# Autodesk Inventor assembly: LR_01
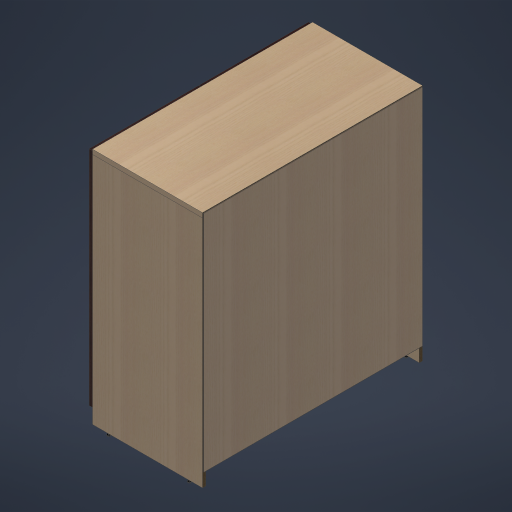
[picture p0: Inventor's stored thumbnail of the model, 512x512]
Saved by Autodesk Inventor 2024.3 (Build 283343000, 343)
## iProperties
Created: 2013-04-03
Part Number: LR_01
Document SubType Name: Assembly
Designer: User
Description: Coat Check
Material Code: Item.FillWorkpiece.Material.Code
Author: User
## Documents named in this file (17)
- C:\W4INV 2024 Design\PROJECTS\Living Room\Coat Check\LR_01.iam
- C:\W4INV 2024 Design\PROJECTS\Samples\Living Room\Coat Check\LR_0108.ipt
- C:\W4INV 2024 Design\PROJECTS\Samples\Living Room\Coat Check\LR_0103.ipt
- C:\W4INV 2024 Design\PROJECTS\Samples\Living Room\Coat Check\LR_0100.ipt
- C:\W4INV 2024 Design\PROJECTS\Samples\Living Room\Coat Check\LR_0102.ipt
- C:\W4INV 2024 Design\PROJECTS\Samples\Living Room\Coat Check\LR_0104.ipt
- C:\W4INV 2024 Design\PROJECTS\Samples\Living Room\Coat Check\LR_0101.ipt
- C:\W4INV 2024 Design\PROJECTS\Samples\Living Room\Coat Check\LR_0105.ipt
- C:\W4INV 2024 Design\PROJECTS\Samples\Living Room\Coat Check\LR_0106.ipt
- C:\W4INV 2024 Design\PROJECTS\Samples\Living Room\Coat Check\LR_0107.ipt
- C:\W4INV 2024 Design\_LIBRARY\Hinges\CONCEALED HINGE\Full Overlay Hinge Wood Screw Cup Wood Screw T18.iam
- C:\W4INV 2024 Design\_LIBRARY\Fixed joints\Minifix joint\MINIFIX D15 v2\Minifix D15 & Dowel L34 & Cap D15 PB T18 LH.ipt
- C:\W4INV 2024 Design\_LIBRARY\Fixed joints\Minifix joint\MINIFIX D15 v2\Minifix D15 & Dowel L34 & Cap D15 PB T18 RH.ipt
- C:\W4INV 2024 Design\_LIBRARY\Supports and legs\Supports\ADJUSTABLE SUPPORT\Support M6 H27 D18 with Bushing SB T18.ipt
- C:\W4INV 2023 Design\LIBRARY\Hinges\CONCEALED HINGE.iam
- C:\W4INV 2023 Design\LIBRARY\Supports and legs\Supports\ADJUSTABLE SUPPORT.ipt
- C:\W4INV 2023 Design\LIBRARY\Fixed joints\Minifix joint\MINIFIX D15 v2.ipt
## Components (29 placed, 13 different names)
1. LR_0108-Top:1 — Mate:46, Mate:48, Mate:50, Mate:52, Mate:54, Mate:56
2. LR_0103-Left Side:1 — Mate:14, Flush:30, Mate:16, Mate:18, Flush:32, Mate:20, Flush:33, Mate:22, Mate:24, Flush:35, Mate:26, Mate:28, Mate:30, Mate:38, Flush:45, Flush:48
3. LR_0100-Right Side:1 — Flush:1, Flush:2, Flush:29, Flush:31, Flush:34, Flush:36, Mate:36, Mate:44, Flush:47, Flush:50
4. LR_0102-Bottom:1 — Flush:37, Flush:40, Flush:41, Flush:44, Mate:58, Mate:60
5. LR_0104-Left Door:1
6. LR_0101-Right Door:1 — Flush:3, Flush:4
7. LR_0105-Back:1
8. LR_0106-Plynth:1
9. LR_0107-Vertical Partition:1 — Flush:46, Flush:49, Flush:51, Flush:52
10. Full Overlay Hinge Wood Screw Cup Wood Screw T18:1 [sub-assembly] — Mate:13, Flush:29, Mate:14
11. Full Overlay Hinge Wood Screw Cup Wood Screw T18:2 [sub-assembly] — Mate:15, Flush:30, Mate:16
12. Full Overlay Hinge Wood Screw Cup Wood Screw T18:3 [sub-assembly] — Mate:17, Flush:31, Mate:18
13. Full Overlay Hinge Wood Screw Cup Wood Screw T18:4 [sub-assembly] — Mate:19, Flush:32, Mate:20
14. Support M6 H27 D18 with Bushing SB T18:6 — Mate:21, Flush:33, Mate:22
15. Support M6 H27 D18 with Bushing SB T18:7 — Mate:23, Flush:34, Mate:24
16. Support M6 H27 D18 with Bushing SB T18:8 — Mate:25, Flush:35, Mate:26
17. Support M6 H27 D18 with Bushing SB T18:9 — Mate:27, Flush:36, Mate:28
18. Minifix D15 & Dowel L34 & Cap D15 PB T18 LH:1 — Mate:29, Mate:30, Flush:37
19. Minifix D15 & Dowel L34 & Cap D15 PB T18 RH:4 — Mate:35, Mate:36, Flush:40
20. Minifix D15 & Dowel L34 & Cap D15 PB T18 RH:5 — Mate:37, Mate:38, Flush:41
21. Minifix D15 & Dowel L34 & Cap D15 PB T18 LH:8 — Mate:43, Mate:44, Flush:44
22. Minifix D15 & Dowel L34 & Cap D15 PB T18 LH:9 — Mate:45, Flush:45, Mate:46
23. Minifix D15 & Dowel L34 & Cap D15 PB T18 RH:10 — Mate:47, Flush:46, Mate:48
24. Minifix D15 & Dowel L34 & Cap D15 PB T18 RH:11 — Mate:49, Flush:47, Mate:50
25. Minifix D15 & Dowel L34 & Cap D15 PB T18 RH:12 — Mate:51, Flush:48, Mate:52
26. Minifix D15 & Dowel L34 & Cap D15 PB T18 LH:13 — Mate:53, Flush:49, Mate:54
27. Minifix D15 & Dowel L34 & Cap D15 PB T18 LH:14 — Mate:55, Flush:50, Mate:56
28. Minifix D15 & Dowel L34 & Cap D15 PB T18 LH:15 — Mate:57, Mate:58, Flush:51
29. Minifix D15 & Dowel L34 & Cap D15 PB T18 RH:16 — Mate:59, Mate:60, Flush:52
## Relationships (64: Mate 40, Flush 24)
- Flush:1 (-80 mm): LR_0100-Right Side:1
- Flush:2 (-80 mm): LR_0100-Right Side:1
- Flush:3 (-100 mm): LR_0101-Right Door:1
- Flush:4 (-100 mm): LR_0101-Right Door:1
- Mate:13: Full Overlay Hinge Wood Screw Cup Wood Screw T18:1
- Flush:29: LR_0100-Right Side:1 ↔ Full Overlay Hinge Wood Screw Cup Wood Screw T18:1
- Mate:14: LR_0103-Left Side:1 ↔ Full Overlay Hinge Wood Screw Cup Wood Screw T18:1
- Mate:15: Full Overlay Hinge Wood Screw Cup Wood Screw T18:2
- Flush:30: LR_0103-Left Side:1 ↔ Full Overlay Hinge Wood Screw Cup Wood Screw T18:2
- Mate:16: LR_0103-Left Side:1 ↔ Full Overlay Hinge Wood Screw Cup Wood Screw T18:2
- Mate:17: Full Overlay Hinge Wood Screw Cup Wood Screw T18:3
- Flush:31: LR_0100-Right Side:1 ↔ Full Overlay Hinge Wood Screw Cup Wood Screw T18:3
- Mate:18: LR_0103-Left Side:1 ↔ Full Overlay Hinge Wood Screw Cup Wood Screw T18:3
- Mate:19: Full Overlay Hinge Wood Screw Cup Wood Screw T18:4
- Flush:32: LR_0103-Left Side:1 ↔ Full Overlay Hinge Wood Screw Cup Wood Screw T18:4
- Mate:20: LR_0103-Left Side:1 ↔ Full Overlay Hinge Wood Screw Cup Wood Screw T18:4
- Mate:21: Support M6 H27 D18 with Bushing SB T18:6
- Flush:33 (9 mm): LR_0103-Left Side:1 ↔ Support M6 H27 D18 with Bushing SB T18:6
- Mate:22 (17.5 mm): LR_0103-Left Side:1 ↔ Support M6 H27 D18 with Bushing SB T18:6
- Mate:23: Support M6 H27 D18 with Bushing SB T18:7
- Flush:34 (9 mm): LR_0100-Right Side:1 ↔ Support M6 H27 D18 with Bushing SB T18:7
- Mate:24 (17.5 mm): LR_0103-Left Side:1 ↔ Support M6 H27 D18 with Bushing SB T18:7
- Mate:25: Support M6 H27 D18 with Bushing SB T18:8
- Flush:35 (9 mm): LR_0103-Left Side:1 ↔ Support M6 H27 D18 with Bushing SB T18:8
- Mate:26 (17.5 mm): LR_0103-Left Side:1 ↔ Support M6 H27 D18 with Bushing SB T18:8
- Mate:27: Support M6 H27 D18 with Bushing SB T18:9
- Flush:36 (9 mm): LR_0100-Right Side:1 ↔ Support M6 H27 D18 with Bushing SB T18:9
- Mate:28 (17.5 mm): LR_0103-Left Side:1 ↔ Support M6 H27 D18 with Bushing SB T18:9
- Mate:29: Minifix D15 & Dowel L34 & Cap D15 PB T18 LH:1
- Mate:30: LR_0103-Left Side:1 ↔ Minifix D15 & Dowel L34 & Cap D15 PB T18 LH:1
- Flush:37 (18 mm): LR_0102-Bottom:1 ↔ Minifix D15 & Dowel L34 & Cap D15 PB T18 LH:1
- Mate:35: Minifix D15 & Dowel L34 & Cap D15 PB T18 RH:4
- Mate:36: LR_0100-Right Side:1 ↔ Minifix D15 & Dowel L34 & Cap D15 PB T18 RH:4
- Flush:40 (18 mm): LR_0102-Bottom:1 ↔ Minifix D15 & Dowel L34 & Cap D15 PB T18 RH:4
- Mate:37: Minifix D15 & Dowel L34 & Cap D15 PB T18 RH:5
- Mate:38: LR_0103-Left Side:1 ↔ Minifix D15 & Dowel L34 & Cap D15 PB T18 RH:5
- Flush:41 (18 mm): LR_0102-Bottom:1 ↔ Minifix D15 & Dowel L34 & Cap D15 PB T18 RH:5
- Mate:43: Minifix D15 & Dowel L34 & Cap D15 PB T18 LH:8
- Mate:44: LR_0100-Right Side:1 ↔ Minifix D15 & Dowel L34 & Cap D15 PB T18 LH:8
- Flush:44 (18 mm): LR_0102-Bottom:1 ↔ Minifix D15 & Dowel L34 & Cap D15 PB T18 LH:8
- Mate:45: Minifix D15 & Dowel L34 & Cap D15 PB T18 LH:9
- Flush:45 (18 mm): LR_0103-Left Side:1 ↔ Minifix D15 & Dowel L34 & Cap D15 PB T18 LH:9
- Mate:46: LR_0108-Top:1 ↔ Minifix D15 & Dowel L34 & Cap D15 PB T18 LH:9
- Mate:47: Minifix D15 & Dowel L34 & Cap D15 PB T18 RH:10
- Flush:46 (18 mm): LR_0107-Vertical Partition:1 ↔ Minifix D15 & Dowel L34 & Cap D15 PB T18 RH:10
- Mate:48: LR_0108-Top:1 ↔ Minifix D15 & Dowel L34 & Cap D15 PB T18 RH:10
- Mate:49: Minifix D15 & Dowel L34 & Cap D15 PB T18 RH:11
- Flush:47 (18 mm): LR_0100-Right Side:1 ↔ Minifix D15 & Dowel L34 & Cap D15 PB T18 RH:11
- Mate:50: LR_0108-Top:1 ↔ Minifix D15 & Dowel L34 & Cap D15 PB T18 RH:11
- Mate:51: Minifix D15 & Dowel L34 & Cap D15 PB T18 RH:12
- Flush:48 (18 mm): LR_0103-Left Side:1 ↔ Minifix D15 & Dowel L34 & Cap D15 PB T18 RH:12
- Mate:52: LR_0108-Top:1 ↔ Minifix D15 & Dowel L34 & Cap D15 PB T18 RH:12
- Mate:53: Minifix D15 & Dowel L34 & Cap D15 PB T18 LH:13
- Flush:49 (18 mm): LR_0107-Vertical Partition:1 ↔ Minifix D15 & Dowel L34 & Cap D15 PB T18 LH:13
- Mate:54: LR_0108-Top:1 ↔ Minifix D15 & Dowel L34 & Cap D15 PB T18 LH:13
- Mate:55: Minifix D15 & Dowel L34 & Cap D15 PB T18 LH:14
- Flush:50 (18 mm): LR_0100-Right Side:1 ↔ Minifix D15 & Dowel L34 & Cap D15 PB T18 LH:14
- Mate:56: LR_0108-Top:1 ↔ Minifix D15 & Dowel L34 & Cap D15 PB T18 LH:14
- Mate:57: Minifix D15 & Dowel L34 & Cap D15 PB T18 LH:15
- Mate:58: LR_0102-Bottom:1 ↔ Minifix D15 & Dowel L34 & Cap D15 PB T18 LH:15
- Flush:51 (18 mm): LR_0107-Vertical Partition:1 ↔ Minifix D15 & Dowel L34 & Cap D15 PB T18 LH:15
- Mate:59: Minifix D15 & Dowel L34 & Cap D15 PB T18 RH:16
- Mate:60: LR_0102-Bottom:1 ↔ Minifix D15 & Dowel L34 & Cap D15 PB T18 RH:16
- Flush:52 (18 mm): LR_0107-Vertical Partition:1 ↔ Minifix D15 & Dowel L34 & Cap D15 PB T18 RH:16
